# Autodesk Inventor assembly: MotorWithClamp
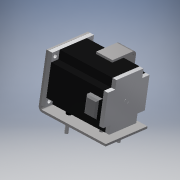
[picture p0: Inventor's stored thumbnail of the model, 180x180]
Saved by Autodesk Inventor 2016 (Build 200138000, 138)
## iProperties
Created: 2017-02-15
Part Number: MotorWithClamp
Document SubType Name: Assembly
Designer: Evan Phil George
Author: Evan Phil George
## Documents named in this file (4)
- C:\Users\Evan Phil George\Desktop\Ball Balancing Robot\TestBenchInventor\SubAssemblies\MotorWithClamp.iam
- C:\Users\Evan Phil George\Desktop\Ball Balancing Robot\TestBenchInventor\SheetMetal\MotorClamptwo.ipt
- C:\Users\Evan Phil George\Desktop\Ball Balancing Robot\TestBenchInventor\SubAssemblies\StepperMotor.iam
- C:\Users\Evan Phil George\Desktop\Ball Balancing Robot\TestBenchInventor\Screw&nuts\Four(mm)20Screw.ipt
## Components (4 placed, 3 different names)
1. MotorClamptwo:1 — Mate:1, Mate:2, Mate:3, Mate:4, Mate:5, Mate:6, Mate:7
2. StepperMotor:1 [sub-assembly] — Mate:1, Mate:2, Mate:3
3. Four(mm)20Screw:1 — Mate:4, Mate:5
4. Four(mm)20Screw:2 — Mate:6, Mate:7
## Relationships (7: Mate 7)
- Mate:1: MotorClamptwo:1 ↔ StepperMotor:1
- Mate:2: MotorClamptwo:1 ↔ StepperMotor:1
- Mate:3: MotorClamptwo:1 ↔ StepperMotor:1
- Mate:4: MotorClamptwo:1 ↔ Four(mm)20Screw:1
- Mate:5: MotorClamptwo:1 ↔ Four(mm)20Screw:1
- Mate:6: MotorClamptwo:1 ↔ Four(mm)20Screw:2
- Mate:7: MotorClamptwo:1 ↔ Four(mm)20Screw:2
